# Autodesk Inventor assembly: Boxer dobry
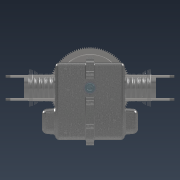
[picture p0: Inventor's stored thumbnail of the model, 180x180]
Saved by Autodesk Inventor 2022 (Build 260153000, 153)
## iProperties
Created: 2023-05-23
Part Number: Boxer dobry
Document SubType Name: Assembly
Designer: wikto
Author: wikto
## Documents named in this file (28)
- C:\Users\wikto\Desktop\Inventor - szkoła\Boxer Garbus\Boxer dobry.iam
- C:\Users\wikto\Desktop\Inventor - szkoła\Boxer Garbus\Blok.ipt
- C:\Users\wikto\Desktop\Inventor - szkoła\Boxer Garbus\Wał korbowy.ipt
- C:\Users\wikto\Desktop\Inventor - szkoła\Boxer Garbus\Łożysko wału korbowego.ipt
- C:\Users\wikto\Desktop\Inventor - szkoła\Boxer Garbus\Łożysko wału korbowego 2.ipt
- C:\Users\wikto\Desktop\Inventor - szkoła\Boxer Garbus\Panewka okrągła.ipt
- C:\Users\wikto\Desktop\Inventor - szkoła\Boxer Garbus\Wałek rozrządu.ipt
- C:\Users\wikto\Desktop\Inventor - szkoła\Boxer Garbus\Panewka wałka rozrzadu koniec.ipt
- C:\Users\wikto\Desktop\Inventor - szkoła\Boxer Garbus\Panewka wałka rozrzadu przod.ipt
- C:\Users\wikto\Desktop\Inventor - szkoła\Boxer Garbus\Panewka wałka rozrzadu srodek.ipt
- C:\Users\wikto\Desktop\Inventor - szkoła\Boxer Garbus\Koło zębate rozrządu\Design Accelerator\Spur Gear15.ipt
- C:\Users\wikto\Desktop\Inventor - szkoła\Boxer Garbus\Koło zębate rozrządu\Design Accelerator\Spur Gear25.ipt
- C:\Users\wikto\Desktop\Inventor - szkoła\Boxer Garbus\Cylinder.ipt
- C:\Users\wikto\Desktop\Inventor - szkoła\Boxer Garbus\Zespół tłoka.iam
- C:\Users\wikto\Desktop\Inventor - szkoła\Boxer Garbus\Korbowód.ipt
- C:\Users\wikto\Desktop\Inventor - szkoła\Boxer Garbus\Blok 2.ipt
- C:\Users\wikto\Desktop\Inventor - szkoła\Boxer Garbus\Pokrywa stopy korbowodu.ipt
- C:\Users\wikto\OneDrive\Documents\Inventor\Content Center Files\R2022\en-US\ISO 14579_2011(E)\ISO 14579 M6x25-8.8.ipt
- C:\Users\wikto\OneDrive\Documents\Inventor\Content Center Files\R2022\en-US\ISO 4162\ISO 4162 - M5 x 50.ipt
- C:\Users\wikto\OneDrive\Documents\Inventor\Content Center Files\R2022\en-US\ISO 4032(2)\ISO 4032 - M5 - ISO.ipt
- C:\Users\wikto\OneDrive\Documents\Inventor\Content Center Files\R2022\en-US\ISO 7089\ISO 7089 - 5 - 140 HV(1).ipt
- C:\Users\wikto\OneDrive\Documents\Inventor\Content Center Files\R2022\en-US\ISO 4017(1)\ISO 4017 - M5 x 16 - ISO.ipt
- C:\Users\wikto\Desktop\Inventor - szkoła\Boxer Garbus\Szpilka głowicy.ipt
- C:\Users\wikto\Desktop\Inventor - szkoła\Boxer Garbus\Koło zamachowe poprawione.ipt
- C:\Users\wikto\OneDrive\Documents\Inventor\Content Center Files\R2022\en-US\ISO 4017(1)\ISO 4017 - M8 x 20 - ISO.ipt
- C:\Users\wikto\Desktop\Inventor - szkoła\Boxer Garbus\Panewka środkowa wału korbowego.ipt
- C:\Users\wikto\Desktop\Inventor - szkoła\Boxer Garbus\Pierścień ustalający.ipt
- C:\Users\wikto\Desktop\Inventor - szkoła\Boxer Garbus\Pierścień klinowy.ipt
## Components (96 placed, 27 different names)
1. Blok:1 — Insert:1, Insert:2, Insert:4, Flush:1, Insert:10, Insert:11, Mate:5, Mate:6, Mate:11, Flush:2, Flush:3, Insert:55, Insert:56, Insert:58, Insert:61, Flush:6, Insert:69, Insert:70, Insert:71, Insert:72
2. Wał korbowy:1 — Mate:1, Mate:2, Insert:7, Insert:8, Insert:12, Insert:13, Insert:16, Insert:17, Insert:22, Insert:23, Insert:24, Insert:25, Mate:66, Mate:67, Mate:68, Insert:67, Insert:68, Rigid:1, Insert:73
3. Łożysko wału korbowego:1 — Insert:8
4. Łożysko wału korbowego 2:1 — Insert:1, Mate:1
5. Panewka okrągła:1 — Insert:2, Mate:2
6. Wałek rozrządu:1 — Insert:5, Insert:6, Mate:3, Insert:21
7. Panewka wałka rozrzadu koniec:1 — Mate:4, Insert:9
8. Panewka wałka rozrzadu koniec:2 — Insert:4, Flush:1, Insert:5, Mate:4, Insert:9
9. Spur Gear1:1 — Insert:7, Rotation:1
10. Spur Gear2:1 — Insert:6, Mate:3, Rotation:1, Mate:60, Mate:61, Mate:70, Mate:71, Mate:72, Mate:73
11. Cylinder:1 — Insert:11, Mate:5, Mate:8
12. Cylinder:2 — Insert:10, Mate:6, Mate:7
13. Zespół tłoka:1 [sub-assembly] — Mate:8, Mate:9
14. Zespół tłoka:2 [sub-assembly] — Mate:7, Mate:10
15. Korbowód:1 — Mate:9, Insert:12, Mate:20, Mate:48, Mate:49, Mate:50, Mate:52, Mate:53, Mate:54
16. Korbowód:2 — Mate:10, Insert:13, Mate:22, Mate:32, Mate:33, Mate:34, Mate:36, Mate:37, Mate:38
17. Blok 2:1 — Mate:11, Flush:2, Flush:3, Insert:14, Insert:15, Mate:12, Mate:13, Insert:18, Flush:4, Insert:20, Flush:5, Insert:26, Insert:27, Insert:28, Insert:29, Insert:30, Insert:31, Insert:32, Insert:33, Insert:34, Insert:35, Insert:36, Insert:37, Insert:38, Insert:47, Insert:48, Insert:49, Insert:50, Insert:51, Insert:52, Insert:53, Insert:54
18. Cylinder:3 — Insert:14, Mate:12, Mate:15
19. Cylinder:4 — Insert:15, Mate:13, Mate:14
20. Zespół tłoka:3 [sub-assembly] — Mate:15, Mate:16
21. Zespół tłoka:4 [sub-assembly] — Mate:14, Mate:17
22. Korbowód:3 — Mate:17, Insert:16, Mate:23, Mate:28, Mate:29, Mate:30, Mate:56, Mate:57, Mate:58
23. Korbowód:4 — Mate:16, Insert:17, Mate:21, Mate:40, Mate:41, Mate:42, Mate:44, Mate:45, Mate:46
24. Panewka wałka rozrzadu srodek:1 — Insert:18, Flush:4, Insert:19, Mate:18
25. Panewka wałka rozrzadu srodek:2 — Insert:19, Mate:18
26. Panewka wałka rozrzadu przod:1 — Insert:21, Mate:19
27. Panewka wałka rozrzadu przod:2 — Insert:20, Flush:5, Mate:19
28. Pokrywa stopy korbowodu:1 — Insert:24, Mate:23, Mate:31, Mate:59
29. Pokrywa stopy korbowodu:2 — Insert:23, Mate:22, Mate:35, Mate:39
30. Pokrywa stopy korbowodu:3 — Insert:25, Mate:20, Mate:51, Mate:55
31. Pokrywa stopy korbowodu:4 — Insert:22, Mate:21, Mate:43, Mate:47
32. Koło zamachowe poprawione:1 — Mate:66, Mate:67, Mate:68, Insert:63, Insert:64, Insert:65, Insert:66
33. Panewka środkowa wału korbowego:1 — Insert:67, Flush:6, Mate:69
34. Panewka środkowa wału korbowego:2 — Mate:69, Insert:68
35. Pierścień ustalający:1 — Rigid:1
36. Pierścień klinowy:1 — Insert:73
37. Szpilka głowicy:1 — Insert:47
38. Szpilka głowicy:2 — Insert:49
39. Szpilka głowicy:3 — Insert:51
40. Szpilka głowicy:4 — Insert:55
41. Szpilka głowicy:5 — Insert:52
42. Szpilka głowicy:6 — Insert:53
43. Szpilka głowicy:7 — Insert:58
44. Szpilka głowicy:8 — Insert:70
45. Szpilka głowicy:9 — Insert:69
46. Szpilka głowicy:10 — Insert:72
47. Szpilka głowicy:11 — Insert:56
48. Szpilka głowicy:12 — Insert:61
49. Szpilka głowicy:13 — Insert:71
50. Szpilka głowicy:14 — Insert:54
51. Szpilka głowicy:15 — Insert:50
52. Szpilka głowicy:16 — Insert:48
53. Screw ISO 14579:2011(E) M6x25-8.8:1 — Insert:26
54. Screw ISO 14579:2011(E) M6x25-8.8:2 — Insert:30
55. Screw ISO 14579:2011(E) M6x25-8.8:3 — Insert:32
56. Screw ISO 14579:2011(E) M6x25-8.8:4 — Insert:33
57. Screw ISO 14579:2011(E) M6x25-8.8:5 — Insert:34
58. Screw ISO 14579:2011(E) M6x25-8.8:6 — Insert:35
59. Screw ISO 14579:2011(E) M6x25-8.8:7 — Insert:36
60. Screw ISO 14579:2011(E) M6x25-8.8:8 — Insert:28
61. Screw ISO 14579:2011(E) M6x25-8.8:9 — Insert:29
62. Screw ISO 14579:2011(E) M6x25-8.8:10 — Insert:31
63. Screw ISO 14579:2011(E) M6x25-8.8:11 — Insert:37
64. Screw ISO 14579:2011(E) M6x25-8.8:12 — Insert:38
65. Screw ISO 14579:2011(E) M6x25-8.8:13 — Insert:27
66. ISO 4162 M5 x 50:2 — Mate:28, Mate:29
67. ISO 7089 5:1 — Mate:30, Mate:31, Insert:39
68. ISO 4032 M5:2 — Insert:39
69. ISO 4162 M5 x 50:3 — Mate:32, Mate:33
70. ISO 7089 5:2 — Mate:34, Mate:35, Insert:40
71. ISO 4032 M5:3 — Insert:40
72. ISO 4162 M5 x 50:4 — Mate:36, Mate:37
73. ISO 7089 5:3 — Mate:38, Mate:39, Insert:41
74. ISO 4032 M5:4 — Insert:41
75. ISO 4162 M5 x 50:5 — Mate:40, Mate:41
76. ISO 7089 5:4 — Mate:42, Mate:43, Insert:42
77. ISO 4032 M5:5 — Insert:42
78. ISO 4162 M5 x 50:6 — Mate:44, Mate:45
79. ISO 7089 5:5 — Mate:46, Mate:47, Insert:43
80. ISO 4032 M5:6 — Insert:43
81. ISO 4162 M5 x 50:7 — Mate:48, Mate:49
82. ISO 7089 5:6 — Mate:50, Mate:51, Insert:44
83. ISO 4032 M5:7 — Insert:44
84. ISO 4162 M5 x 50:8 — Mate:52, Mate:53
85. ISO 7089 5:7 — Mate:54, Mate:55, Insert:45
86. ISO 4032 M5:8 — Insert:45
87. ISO 4162 M5 x 50:9 — Mate:56, Mate:57
88. ISO 7089 5:8 — Mate:58, Mate:59, Insert:46
89. ISO 4032 M5:9 — Insert:46
90. ISO 4017 M5 x 16:3 — Mate:72, Mate:73
91. ISO 4017 M5 x 16:2 — Mate:70, Mate:71
92. ISO 4017 M5 x 16:1 — Mate:60, Mate:61
93. ISO 4017 M8 x 20:1 — Insert:64
94. ISO 4017 M8 x 20:2 — Insert:65
95. ISO 4017 M8 x 20:3 — Insert:66
96. ISO 4017 M8 x 20:4 — Insert:63
## Relationships (141: Insert 68, Mate 65, Flush 6, RelateRotation 1, WeldJoint 1)
- Insert:1: Blok:1 ↔ Łożysko wału korbowego 2:1
- Mate:1: Wał korbowy:1 ↔ Łożysko wału korbowego 2:1
- Insert:2: Blok:1 ↔ Panewka okrągła:1
- Mate:2: Wał korbowy:1 ↔ Panewka okrągła:1
- Insert:4: Blok:1 ↔ Panewka wałka rozrzadu koniec:2
- Flush:1: Blok:1 ↔ Panewka wałka rozrzadu koniec:2
- Insert:5: Wałek rozrządu:1 ↔ Panewka wałka rozrzadu koniec:2
- Insert:6: Wałek rozrządu:1 ↔ Spur Gear2:1
- Mate:3: Wałek rozrządu:1 ↔ Spur Gear2:1
- Insert:7: Wał korbowy:1 ↔ Spur Gear1:1
- Insert:8: Wał korbowy:1 ↔ Łożysko wału korbowego:1
- Rotation:1 [RelateRotation] (2 ul): Spur Gear1:1 ↔ Spur Gear2:1
- Mate:4: Panewka wałka rozrzadu koniec:1 ↔ Panewka wałka rozrzadu koniec:2
- Insert:9: Panewka wałka rozrzadu koniec:1 ↔ Panewka wałka rozrzadu koniec:2
- Insert:10: Blok:1 ↔ Cylinder:2
- Insert:11: Blok:1 ↔ Cylinder:1
- Mate:5: Blok:1 ↔ Cylinder:1
- Mate:6: Blok:1 ↔ Cylinder:2
- Mate:7: Cylinder:2 ↔ Zespół tłoka:2
- Mate:8: Cylinder:1 ↔ Zespół tłoka:1
- Mate:9: Zespół tłoka:1 ↔ Korbowód:1
- Mate:10: Zespół tłoka:2 ↔ Korbowód:2
- Insert:12: Wał korbowy:1 ↔ Korbowód:1
- Insert:13: Wał korbowy:1 ↔ Korbowód:2
- Mate:11: Blok:1 ↔ Blok 2:1
- Flush:2: Blok:1 ↔ Blok 2:1
- Flush:3: Blok:1 ↔ Blok 2:1
- Insert:14: Blok 2:1 ↔ Cylinder:3
- Insert:15: Blok 2:1 ↔ Cylinder:4
- Mate:12: Blok 2:1 ↔ Cylinder:3
- Mate:13: Blok 2:1 ↔ Cylinder:4
- Mate:14: Cylinder:4 ↔ Zespół tłoka:4
- Mate:15: Cylinder:3 ↔ Zespół tłoka:3
- Mate:16: Zespół tłoka:3 ↔ Korbowód:4
- Mate:17: Zespół tłoka:4 ↔ Korbowód:3
- Insert:16: Wał korbowy:1 ↔ Korbowód:3
- Insert:17: Wał korbowy:1 ↔ Korbowód:4
- Insert:18: Blok 2:1 ↔ Panewka wałka rozrzadu srodek:1
- Flush:4: Blok 2:1 ↔ Panewka wałka rozrzadu srodek:1
- Insert:19: Panewka wałka rozrzadu srodek:1 ↔ Panewka wałka rozrzadu srodek:2
- Mate:18: Panewka wałka rozrzadu srodek:1 ↔ Panewka wałka rozrzadu srodek:2
- Insert:20: Blok 2:1 ↔ Panewka wałka rozrzadu przod:2
- Flush:5: Blok 2:1 ↔ Panewka wałka rozrzadu przod:2
- Insert:21: Wałek rozrządu:1 ↔ Panewka wałka rozrzadu przod:1
- Mate:19: Panewka wałka rozrzadu przod:1 ↔ Panewka wałka rozrzadu przod:2
- Insert:22: Wał korbowy:1 ↔ Pokrywa stopy korbowodu:4
- Insert:23: Wał korbowy:1 ↔ Pokrywa stopy korbowodu:2
- Insert:24: Wał korbowy:1 ↔ Pokrywa stopy korbowodu:1
- Insert:25: Wał korbowy:1 ↔ Pokrywa stopy korbowodu:3
- Mate:20: Korbowód:1 ↔ Pokrywa stopy korbowodu:3
- Mate:21: Korbowód:4 ↔ Pokrywa stopy korbowodu:4
- Mate:22: Korbowód:2 ↔ Pokrywa stopy korbowodu:2
- Mate:23: Korbowód:3 ↔ Pokrywa stopy korbowodu:1
- Insert:26: Blok 2:1 ↔ Screw ISO 14579:2011(E) M6x25-8.8:1
- Insert:27: Blok 2:1 ↔ Screw ISO 14579:2011(E) M6x25-8.8:13
- Insert:28: Blok 2:1 ↔ Screw ISO 14579:2011(E) M6x25-8.8:8
- Insert:29: Blok 2:1 ↔ Screw ISO 14579:2011(E) M6x25-8.8:9
- Insert:30: Blok 2:1 ↔ Screw ISO 14579:2011(E) M6x25-8.8:2
- Insert:31: Blok 2:1 ↔ Screw ISO 14579:2011(E) M6x25-8.8:10
- Insert:32: Blok 2:1 ↔ Screw ISO 14579:2011(E) M6x25-8.8:3
- Insert:33: Blok 2:1 ↔ Screw ISO 14579:2011(E) M6x25-8.8:4
- Insert:34: Blok 2:1 ↔ Screw ISO 14579:2011(E) M6x25-8.8:5
- Insert:35: Blok 2:1 ↔ Screw ISO 14579:2011(E) M6x25-8.8:6
- Insert:36: Blok 2:1 ↔ Screw ISO 14579:2011(E) M6x25-8.8:7
- Insert:37: Blok 2:1 ↔ Screw ISO 14579:2011(E) M6x25-8.8:11
- Insert:38: Blok 2:1 ↔ Screw ISO 14579:2011(E) M6x25-8.8:12
- Mate:28: Korbowód:3 ↔ ISO 4162 M5 x 50:2
- Mate:29: Korbowód:3 ↔ ISO 4162 M5 x 50:2
- Mate:30: Korbowód:3 ↔ ISO 7089 5:1
- Mate:31: Pokrywa stopy korbowodu:1 ↔ ISO 7089 5:1
- Insert:39: ISO 7089 5:1 ↔ ISO 4032 M5:2
- Mate:32: Korbowód:2 ↔ ISO 4162 M5 x 50:3
- Mate:33: Korbowód:2 ↔ ISO 4162 M5 x 50:3
- Mate:34: Korbowód:2 ↔ ISO 7089 5:2
- Mate:35: Pokrywa stopy korbowodu:2 ↔ ISO 7089 5:2
- Insert:40: ISO 7089 5:2 ↔ ISO 4032 M5:3
- Mate:36: Korbowód:2 ↔ ISO 4162 M5 x 50:4
- Mate:37: Korbowód:2 ↔ ISO 4162 M5 x 50:4
- Mate:38: Korbowód:2 ↔ ISO 7089 5:3
- Mate:39: Pokrywa stopy korbowodu:2 ↔ ISO 7089 5:3
- Insert:41: ISO 7089 5:3 ↔ ISO 4032 M5:4
- Mate:40: Korbowód:4 ↔ ISO 4162 M5 x 50:5
- Mate:41: Korbowód:4 ↔ ISO 4162 M5 x 50:5
- Mate:42: Korbowód:4 ↔ ISO 7089 5:4
- Mate:43: Pokrywa stopy korbowodu:4 ↔ ISO 7089 5:4
- Insert:42: ISO 7089 5:4 ↔ ISO 4032 M5:5
- Mate:44: Korbowód:4 ↔ ISO 4162 M5 x 50:6
- Mate:45: Korbowód:4 ↔ ISO 4162 M5 x 50:6
- Mate:46: Korbowód:4 ↔ ISO 7089 5:5
- Mate:47: Pokrywa stopy korbowodu:4 ↔ ISO 7089 5:5
- Insert:43: ISO 7089 5:5 ↔ ISO 4032 M5:6
- Mate:48: Korbowód:1 ↔ ISO 4162 M5 x 50:7
- Mate:49: Korbowód:1 ↔ ISO 4162 M5 x 50:7
- Mate:50: Korbowód:1 ↔ ISO 7089 5:6
- Mate:51: Pokrywa stopy korbowodu:3 ↔ ISO 7089 5:6
- Insert:44: ISO 7089 5:6 ↔ ISO 4032 M5:7
- Mate:52: Korbowód:1 ↔ ISO 4162 M5 x 50:8
- Mate:53: Korbowód:1 ↔ ISO 4162 M5 x 50:8
- Mate:54: Korbowód:1 ↔ ISO 7089 5:7
- Mate:55: Pokrywa stopy korbowodu:3 ↔ ISO 7089 5:7
- Insert:45: ISO 7089 5:7 ↔ ISO 4032 M5:8
- Mate:56: Korbowód:3 ↔ ISO 4162 M5 x 50:9
- Mate:57: Korbowód:3 ↔ ISO 4162 M5 x 50:9
- Mate:58: Korbowód:3 ↔ ISO 7089 5:8
- Mate:59: Pokrywa stopy korbowodu:1 ↔ ISO 7089 5:8
- Insert:46: ISO 7089 5:8 ↔ ISO 4032 M5:9
- Mate:60: Spur Gear2:1 ↔ ISO 4017 M5 x 16:1
- Mate:61: Spur Gear2:1 ↔ ISO 4017 M5 x 16:1
- Insert:47: Blok 2:1 ↔ Szpilka głowicy:1
- Insert:48: Blok 2:1 ↔ Szpilka głowicy:16
- Insert:49: Blok 2:1 ↔ Szpilka głowicy:2
- Insert:50: Blok 2:1 ↔ Szpilka głowicy:15
- Insert:51: Blok 2:1 ↔ Szpilka głowicy:3
- Insert:52: Blok 2:1 ↔ Szpilka głowicy:5
- Insert:53: Blok 2:1 ↔ Szpilka głowicy:6
- Insert:54: Blok 2:1 ↔ Szpilka głowicy:14
- Insert:55: Blok:1 ↔ Szpilka głowicy:4
- Insert:56: Blok:1 ↔ Szpilka głowicy:11
- Insert:58: Blok:1 ↔ Szpilka głowicy:7
- Insert:61: Blok:1 ↔ Szpilka głowicy:12
- Mate:66: Wał korbowy:1 ↔ Koło zamachowe poprawione:1
- Mate:67: Wał korbowy:1 ↔ Koło zamachowe poprawione:1
- Mate:68: Wał korbowy:1 ↔ Koło zamachowe poprawione:1
- Insert:63: Koło zamachowe poprawione:1 ↔ ISO 4017 M8 x 20:4
- Insert:64: Koło zamachowe poprawione:1 ↔ ISO 4017 M8 x 20:1
- Insert:65: Koło zamachowe poprawione:1 ↔ ISO 4017 M8 x 20:2
- Insert:66: Koło zamachowe poprawione:1 ↔ ISO 4017 M8 x 20:3
- Insert:67: Wał korbowy:1 ↔ Panewka środkowa wału korbowego:1
- Flush:6: Blok:1 ↔ Panewka środkowa wału korbowego:1
- Mate:69: Panewka środkowa wału korbowego:1 ↔ Panewka środkowa wału korbowego:2
- Insert:68: Wał korbowy:1 ↔ Panewka środkowa wału korbowego:2
- Insert:69: Blok:1 ↔ Szpilka głowicy:9
- Insert:70: Blok:1 ↔ Szpilka głowicy:8
- Insert:71: Blok:1 ↔ Szpilka głowicy:13
- Insert:72: Blok:1 ↔ Szpilka głowicy:10
- Rigid:1 [WeldJoint]: Wał korbowy:1 ↔ Pierścień ustalający:1
- Insert:73: Wał korbowy:1 ↔ Pierścień klinowy:1
- Mate:70: Spur Gear2:1 ↔ ISO 4017 M5 x 16:2
- Mate:71: Spur Gear2:1 ↔ ISO 4017 M5 x 16:2
- Mate:72: Spur Gear2:1 ↔ ISO 4017 M5 x 16:3
- Mate:73: Spur Gear2:1 ↔ ISO 4017 M5 x 16:3
